# Autodesk Inventor assembly: Base
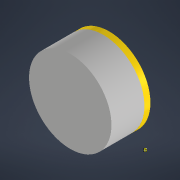
[picture p0: Inventor's stored thumbnail of the model, 180x180]
Saved by Autodesk Inventor 2021 (Build 250183000, 183)
## iProperties
Created: 2022-08-30
Part Number: Base
Document SubType Name: Assembly
Designer: MicnedSQ
Author: MicnedSQ
## Documents named in this file (9)
- C:\Users\MicnedSQ\Desktop\RobotArmV1\Base\Base.iam
- C:\Users\MicnedSQ\Desktop\RobotArmV1\Base\Część8.ipt
- C:\Users\MicnedSQ\Desktop\RobotArmV1\Bearing 25x32x4\AIS2021\SKF_W 61705-2RS1.iam
- C:\Users\MicnedSQ\Desktop\RobotArmV1\Base\Rotor.ipt
- C:\Users\MicnedSQ\Desktop\RobotArmV1\Base\RotorShaft.iam
- C:\Users\MicnedSQ\Desktop\RobotArmV1\Base\OutputShaft.ipt
- C:\Users\MicnedSQ\Desktop\RobotArmV1\Base\OutputShaft2.ipt
- C:\Users\MicnedSQ\Desktop\RobotArmV1\Base\Top.ipt
- C:\Users\MicnedSQ\Desktop\RobotArmV1\Base\Bottom.ipt
## Components (10 placed, 8 different names)
1. Część8:1 — Sztywne:1, Sztywne:3
2. SKF_W 61705-2RS1:1 [sub-assembly] — Sztywne:1, Obrotowe:1
3. RotorShaft:1 [sub-assembly] — Obrotowe:1, Obrotowe:2, Obrót:1, Obrotowe:5
4. SKF_W 61705-2RS1:2 [sub-assembly] — Obrotowe:2, Obrotowe:3
5. Rotor:1 — Obrotowe:3, Obrót:1
6. SKF_W 61705-2RS1:3 [sub-assembly] — Obrotowe:4, Obrotowe:5
7. OutputShaft:1 — Obrotowe:4, Sztywne:2
8. OutputShaft2:1 — Sztywne:2
9. Top:1 — Sztywne:3, Sztywne:4
10. Bottom:1 — Sztywne:4
## Relationships (10: RevoluteJoint 5, WeldJoint 4, RelateRotation 1)
- Sztywne:1 [WeldJoint]: Część8:1 ↔ SKF_W 61705-2RS1:1
- Obrotowe:1 [RevoluteJoint]: SKF_W 61705-2RS1:1 ↔ RotorShaft:1
- Obrotowe:2 [RevoluteJoint]: RotorShaft:1 ↔ SKF_W 61705-2RS1:2
- Obrotowe:3 [RevoluteJoint]: SKF_W 61705-2RS1:2 ↔ Rotor:1
- Obrót:1 [RelateRotation] (0.0526 ul): RotorShaft:1 ↔ Rotor:1
- Obrotowe:4 [RevoluteJoint]: SKF_W 61705-2RS1:3 ↔ OutputShaft:1
- Obrotowe:5 [RevoluteJoint]: RotorShaft:1 ↔ SKF_W 61705-2RS1:3
- Sztywne:2 [WeldJoint]: OutputShaft:1 ↔ OutputShaft2:1
- Sztywne:3 [WeldJoint]: Część8:1 ↔ Top:1
- Sztywne:4 [WeldJoint]: Top:1 ↔ Bottom:1
